# Autodesk Inventor assembly: Motor
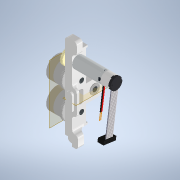
[picture p0: Inventor's stored thumbnail of the model, 180x180]
Saved by Autodesk Inventor 2022 (Build 260153000, 153)
## iProperties
Created: 2021-09-24
Part Number: Motor
Document SubType Name: Assembly
Designer: shiok
Mass: 31.1386 g
Surface Area: 214.594 cm^2
Volume: 14.9157 cm^3
Density: 2.08764 g/cm^3
Author: shiok
## Documents named in this file (10)
- C:\Users\Yazawa\Documents\GitHub\murakumo\inventor\Motor.iam
- C:\Users\Yazawa\Documents\GitHub\murakumo\inventor\maxon DCX 10L.iam
- C:\Users\Yazawa\Documents\GitHub\murakumo\inventor\Tire.iam
- C:\Users\Yazawa\Documents\GitHub\murakumo\inventor\piniongear_41_middle.ipt
- C:\Users\Yazawa\Documents\GitHub\murakumo\inventor\piniongear_41_src.ipt
- C:\Users\Yazawa\Documents\GitHub\murakumo\inventor\shaft_short.ipt
- C:\Users\Yazawa\Documents\GitHub\murakumo\inventor\MotorBracketv2.ipt
- C:\Users\Yazawa\Documents\GitHub\murakumo\inventor\FL674ZZ_MIR.ipt
- C:\Users\Yazawa\Documents\GitHub\murakumo\inventor\Motor\デザイン アクセラレータ\平歯車3.iam
- C:\Users\Yazawa\Documents\GitHub\murakumo\inventor\Motor\デザイン アクセラレータ\平歯車4.iam
## Components (11 placed, 8 different names)
1. Tire:1 [sub-assembly] — メイト:12, フラッシュ:2, 対称度:1
2. MotorBracketv2:1 — メイト:1, メイト:2, メイト:3, メイト:4, メイト:8, メイト:10, メイト:11, メイト:12, メイト:13, フラッシュ:5
3. Tire:2 [sub-assembly] — メイト:11, フラッシュ:1, フラッシュ:3, 対称度:1, 対称度:2
4. maxon DCX 10L:1 [sub-assembly] — メイト:8, メイト:9, メイト:10, 対称度:2
5. FL674ZZ_MIR:1 — メイト:3, メイト:4
6. FL674ZZ_MIR:2 — メイト:1, メイト:2, メイト:5, フラッシュ:4
7. piniongear_41_middle:1 — 挿入:6, フラッシュ:1, フラッシュ:2
8. piniongear_41_src:1 — メイト:9, フラッシュ:3
9. shaft_short:1 — 挿入:6, メイト:5, フラッシュ:4
10. 平歯車:1 [sub-assembly]
11. 平歯車:2 [sub-assembly]
## Relationships (20: Mate 12, Flush 5, Symmetry 2, Insert 1)
- 挿入:6 [Insert]: piniongear_41_middle:1 ↔ shaft_short:1
- メイト:1 [Mate]: MotorBracketv2:1 ↔ FL674ZZ_MIR:2
- メイト:2 [Mate]: MotorBracketv2:1 ↔ FL674ZZ_MIR:2
- メイト:3 [Mate]: MotorBracketv2:1 ↔ FL674ZZ_MIR:1
- メイト:4 [Mate]: MotorBracketv2:1 ↔ FL674ZZ_MIR:1
- メイト:5 [Mate]: FL674ZZ_MIR:2 ↔ shaft_short:1
- メイト:8 [Mate]: MotorBracketv2:1 ↔ maxon DCX 10L:1
- メイト:9 [Mate]: maxon DCX 10L:1 ↔ piniongear_41_src:1
- メイト:10 [Mate]: MotorBracketv2:1 ↔ maxon DCX 10L:1
- メイト:11 [Mate]: MotorBracketv2:1 ↔ Tire:2
- メイト:12 [Mate]: Tire:1 ↔ MotorBracketv2:1
- フラッシュ:1 [Flush]: Tire:2 ↔ piniongear_41_middle:1
- フラッシュ:2 [Flush]: Tire:1 ↔ piniongear_41_middle:1
- フラッシュ:3 [Flush]: Tire:2 ↔ piniongear_41_src:1
- フラッシュ:4 [Flush]: FL674ZZ_MIR:2 ↔ shaft_short:1
- メイト:13 [Mate]: MotorBracketv2:1
- 対称度:1 [Symmetry]: Tire:1 ↔ Tire:2
- フラッシュ:5 [Flush]: MotorBracketv2:1
- 対称度:2 [Symmetry]: Tire:2 ↔ maxon DCX 10L:1
- メイト:14 [Mate]
